# Autodesk Inventor assembly: Jose_Ensamble_Set_Sobre_Robot
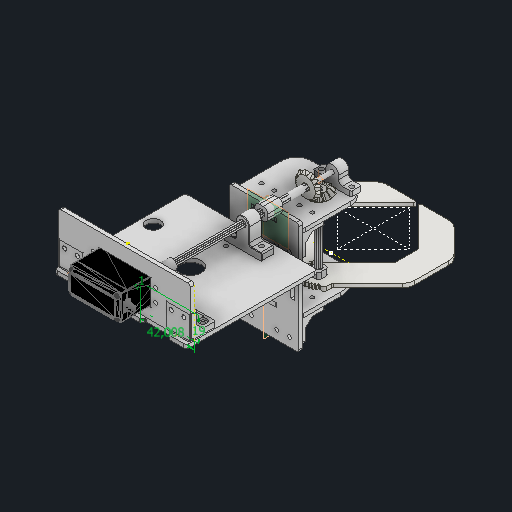
[picture p0: Inventor's stored thumbnail of the model, 512x512]
Saved by Autodesk Inventor 2027 (Build 310192000, 192)
## iProperties
Created: 2025-10-21
Part Number: Jose_Ensamble_Set_Sobre_Robot
Document SubType Name: Assembly
Designer: brene
Author: brene
## Documents named in this file (5)
- C:\Users\06aar\OneDrive\Programas\GitHub\Atta-Bot-STEM\Chasis\1. Diseño V3.0\SetHerramientas\PiezasSTD\Jose_Ensamble_Set_Sobre_Robot.iam
- C:\Users\06aar\OneDrive\Programas\GitHub\Atta-Bot-STEM\Chasis\1. Diseño V3.0\SetHerramientas\PiezasSTD\EnsambleGarraSTD.iam
- C:\Users\06aar\OneDrive\Programas\GitHub\Atta-Bot-STEM\Chasis\1. Diseño V3.0\SetHerramientas\PiezasSTD\DistanciaSpacer3mm.ipt
- C:\Users\06aar\OneDrive\Programas\GitHub\Atta-Bot-STEM\Chasis\1. Diseño V3.0\SetHerramientas\PiezasSTD\EnsambleMotor\EnsambleBaseMotor.iam
- C:\Users\06aar\OneDrive\Programas\GitHub\Atta-Bot-STEM\Chasis\1. Diseño V3.0\SetHerramientas\PiezasSTD\EnsambleMotor\EjeMotor.ipt
## Components (4 placed, 4 different names)
1. EnsambleGarraSTD:1 [sub-assembly] — Mate:293, Mate:294, Flush:222
2. DistanciaSpacer3mm:1 — Mate:293
3. EjeMotor:1 — Flush:222
4. EnsambleBaseMotor_Mediciones [sub-assembly] — Angle:7, Angle:8
## Relationships (5: Mate 2, Angle 2, Flush 1)
- Mate:293: EnsambleGarraSTD:1 ↔ DistanciaSpacer3mm:1
- Mate:294: EnsambleGarraSTD:1
- Flush:222: EnsambleGarraSTD:1 ↔ EjeMotor:1
- Angle:7 (180 deg): EnsambleBaseMotor_Mediciones
- Angle:8 (180 deg): EnsambleBaseMotor_Mediciones
